# Autodesk Inventor assembly: Piston
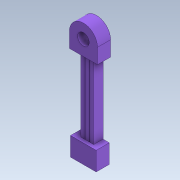
[picture p0: Inventor's stored thumbnail of the model, 180x180]
Saved by Autodesk Inventor 2020 (Build 240168000, 168)
## iProperties
Created: 2020-10-17
Part Number: Piston
Document SubType Name: Assembly
Designer: Turing
Author: Turing
## Documents named in this file (3)
- D:\Hexapod3DPrint\Piston.iam
- D:\Hexapod3DPrint\PistonBot.ipt
- D:\Hexapod3DPrint\PistonTop.ipt
## Components (2 placed, 2 different names)
1. PistonBot:1 — Rigid:1
2. PistonTop:1 — Rigid:1
## Relationships (1: WeldJoint 1)
- Rigid:1 [WeldJoint]: PistonBot:1 ↔ PistonTop:1
